# Autodesk Inventor assembly: chassis
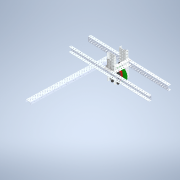
[picture p0: Inventor's stored thumbnail of the model, 180x180]
Saved by Autodesk Inventor 2021 (Build 250183000, 183)
## iProperties
Created: 2020-05-02
Part Number: chassis
Document SubType Name: Assembly
Designer: ajcar
Author: ajcar
## Documents named in this file (4)
- C:\Users\ajcar\Documents\vex_cad\chassis\chassis.iam
- C:\Users\ajcar\Documents\vex_cad\lib\Team 7479 Solidworks Library\Structure\C-Channel\C-Channel 1x2x1x35.ipt
- C:\Users\ajcar\Documents\vex_cad\tracking_wheels\tracking_wheels_v1.iam
- C:\Users\ajcar\Documents\vex_cad\lib\Team 7479 Solidworks Library\Structure\Misc\Angle Gusset.ipt
## Components (6 placed, 3 different names)
1. C-Channel 1x2x1x35:1 — Insert:6
2. C-Channel 1x2x1x35:2 — Angle:2, Mate:1, Angle:3, Mate:2, Angle:4, Insert:5, Insert:6
3. C-Channel 1x2x1x35:3 — Insert:4
4. tracking_wheels_v1:1 [sub-assembly] — Angle:2
5. Angle Gusset:1 — Mate:2, Angle:4, Insert:5
6. Angle Gusset:2 — Mate:1, Angle:3, Insert:4
## Relationships (11: Insert 5, Angle 4, Mate 2)
- [Angle] (90 deg): C-Channel 1x2x1x35:1 ↔ C-Channel 1x2x1x35:2
- [Insert]: C-Channel 1x2x1x35:1 ↔ C-Channel 1x2x1x35:3
- [Insert]: C-Channel 1x2x1x35:1 ↔ C-Channel 1x2x1x35:3
- Angle:2 (0 deg): C-Channel 1x2x1x35:2 ↔ tracking_wheels_v1:1
- Mate:1: C-Channel 1x2x1x35:2 ↔ Angle Gusset:2
- Angle:3 (0 deg): C-Channel 1x2x1x35:2 ↔ Angle Gusset:2
- Insert:4: C-Channel 1x2x1x35:3 ↔ Angle Gusset:2
- Mate:2: C-Channel 1x2x1x35:2 ↔ Angle Gusset:1
- Angle:4 (0 deg): C-Channel 1x2x1x35:2 ↔ Angle Gusset:1
- Insert:5: C-Channel 1x2x1x35:2 ↔ Angle Gusset:1
- Insert:6: C-Channel 1x2x1x35:1 ↔ C-Channel 1x2x1x35:2
## Named parameters: d0_d1 = 90 deg, d1_d3 = 0 mm
